# Autodesk Inventor assembly: ASY MSC 900.7 BASE FRAME TRANSVERSE 1
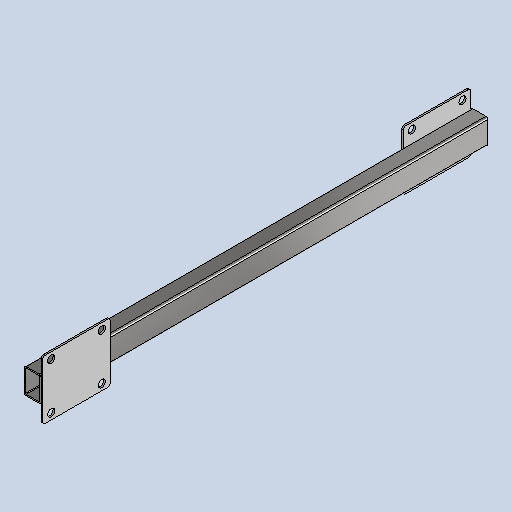
[picture p0: Inventor's stored thumbnail of the model, 512x512]
Saved by Autodesk Inventor 2025 (Build 290162010, 162A)
## iProperties
Created: 2024-09-11
Part Number: ASY MSC 900.7 BASE FRAME TRANSVERSE 1
Document SubType Name: Assembly
Designer: admin
Stock Number: МОО 900.7 связь 1
Author: admin
## Documents named in this file (3)
- C:\Users\admin\YandexDisk-badmisterfox\домашниий пк\Inventor\Manturovo\Manturovo_Se-clar\ASY 940 linkage.iam
- C:\Users\admin\YandexDisk-badmisterfox\домашниий пк\Inventor\Manturovo\Manturovo_Se-clar\MSC 908 transverse pillar plate.ipt
- C:\Users\admin\YandexDisk-badmisterfox\домашниий пк\Inventor\Manturovo\Manturovo_Se-clar\ISO 657_14 - 60x40x3 - 1000.ipt
## Components (3 placed, 2 different names)
1. MSC 908 transverse pillar plate.ipt:1
2. MSC 908 transverse pillar plate.ipt:2
3. ISO 657_14 - 60x40x3 - 1000.ipt:1
## Relationships (2: WeldJoint 2)
- [WeldJoint]: MSC 908 transverse pillar plate.ipt:2 ↔ ISO 657_14 - 60x40x3 - 1000.ipt:1
- [WeldJoint]: MSC 908 transverse pillar plate.ipt:1 ↔ ISO 657_14 - 60x40x3 - 1000.ipt:1
